# Autodesk Inventor assembly: Bottom_Assembly
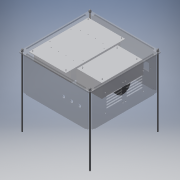
[picture p0: Inventor's stored thumbnail of the model, 180x180]
Saved by Autodesk Inventor 2016 (Build 200138000, 138)
## iProperties
Created: 2018-05-12
Part Number: Bottom_Assembly
Document SubType Name: Assembly
Designer: Phil Erle
Author: Phil Erle
## Documents named in this file (29)
- C:\Users\Phil Erle\Desktop\Adrastea\Bottom_Assembly.iam
- C:\Users\Phil Erle\Desktop\Adrastea\bottom.ipt
- C:\Users\Phil Erle\Desktop\Adrastea\Heatsink.ipt
- C:\Users\Phil Erle\Desktop\Adrastea\Elektronik_Gehäuse.ipt
- C:\Users\Phil Erle\Desktop\Adrastea\GT175DA120U.ipt
- C:\Users\Phil Erle\Desktop\Adrastea\SeitenUntenHinten.ipt
- C:\Users\Phil Erle\Desktop\Adrastea\SeitenUnten.ipt
- C:\Users\Phil Erle\Desktop\Adrastea\SeitenUntenVorne.ipt
- C:\Users\Phil Erle\Desktop\Adrastea\SeitenOben.ipt
- C:\Users\Phil Erle\Desktop\Adrastea\mid.ipt
- C:\Users\Phil Erle\Desktop\Adrastea\Main.ipt
- C:\Users\Phil Erle\Desktop\Adrastea\Primary.ipt
- C:\Users\Phil Erle\Desktop\Adrastea\Normteile\Muttern\din1587-m5x0_8ricu3.ipt
- C:\Users\Phil Erle\Desktop\Adrastea\Seconday_End_Bottom.ipt
- C:\Users\Phil Erle\Desktop\Adrastea\M5 Gewindestange.ipt
- C:\Users\Phil Erle\Desktop\Adrastea\Normteile\Muttern\mutter_din934_m5-6.ipt
- C:\Users\Phil Erle\Desktop\Adrastea\Secondary.ipt
- C:\Users\Phil Erle\Desktop\Adrastea\TopLoad.ipt
- C:\Users\Phil Erle\Desktop\Adrastea\Seconday_End_Top.ipt
- C:\Users\Phil Erle\Desktop\Adrastea\M6 Gewindestange.ipt
- C:\Users\Phil Erle\Desktop\Adrastea\top.ipt
- C:\Users\Phil Erle\Desktop\Adrastea\Coil.ipt
- C:\Users\Phil Erle\Desktop\Adrastea\primary_holder.ipt
- C:\Users\Phil Erle\Desktop\Adrastea\IGBT_Platine.ipt
- C:\Users\Phil Erle\Desktop\Adrastea\Cap_Holder_1.ipt
- C:\Users\Phil Erle\Desktop\Adrastea\Cap.ipt
- C:\Users\Phil Erle\Desktop\Adrastea\Abstandshalter_10mm_M4.ipt
- C:\Users\Phil Erle\Desktop\Adrastea\CU5.ipt
- C:\Users\Phil Erle\Desktop\Adrastea\Snubber.ipt
## Components (50 placed, 28 different names)
1. bottom:1 — Mate:1, Mate:2, Flush:1, Mate:3, Mate:4, Mate:5, Mate:6, Mate:7, Mate:8, Mate:21, Mate:24, Mate:25, Mate:27, Mate:31, Mate:32, Mate:36, Mate:37, Mate:38, Mate:39, Mate:40, Mate:41, Mate:60, Mate:61, Mate:62, Mate:63, Mate:64, Mate:65, Mate:66, Mate:67, Mate:68, Mate:69, Mate:70, Mate:71, Flush:2, Flush:3, Flush:4, Flush:5
2. Heatsink:1 — Mate:3, Mate:4, Mate:5, Mate:9, Mate:10, Mate:11, Mate:12, Mate:13, Mate:14, Mate:15, Mate:16, Mate:17, Mate:18, Mate:19, Mate:20, Mate:106, Mate:107
3. Elektronik_Gehäuse:1 — Mate:6, Mate:7, Mate:8
4. GT175DA120U:1 — Mate:9, Mate:16, Mate:20, Mate:103, Mate:104, Mate:105, Mate:109, Mate:110, Mate:111
5. GT175DA120U:2 — Mate:10, Mate:14, Mate:19
6. GT175DA120U:3 — Mate:11, Mate:15, Mate:18
7. GT175DA120U:4 — Mate:12, Mate:13, Mate:17
8. SeitenUntenHinten:1 — Mate:21, Mate:27, Mate:31, Mate:34
9. SeitenUnten:1 — Mate:36, Mate:37, Mate:38
10. SeitenUnten:2 — Mate:24, Mate:25, Mate:32, Mate:43
11. SeitenUntenVorne:1 — Mate:39, Mate:40, Mate:41, Mate:42, Mate:44
12. SeitenOben:1 — Mate:45, Mate:51, Mate:56, Mate:59
13. SeitenOben:2 — Mate:46, Mate:52, Mate:53, Mate:58
14. SeitenOben:3 — Mate:48, Mate:49, Mate:55, Mate:57
15. SeitenOben:4 — Mate:47, Mate:50, Mate:54
16. mid:1 — Mate:34, Mate:42, Mate:43, Mate:44, Mate:45, Mate:46, Mate:47, Mate:48, Mate:49, Mate:50, Mate:51, Mate:52, Mate:53, Mate:54, Mate:55, Mate:56
17. Main:1 — Mate:57, Mate:58, Mate:59, Mate:72, Mate:73, Mate:75, Mate:76, Mate:77, Mate:85, Mate:86, Mate:87, Mate:88, Mate:92
18. Primary:1 — Mate:89, Mate:90, Mate:91
19. din1587-m5x0_8ricu3:1 — Mate:62, Mate:65
20. din1587-m5x0_8ricu3:2 — Mate:63, Mate:67
21. din1587-m5x0_8ricu3:3 — Mate:60, Mate:66
22. din1587-m5x0_8ricu3:4 — Mate:61, Mate:64
23. Seconday_End_Bottom:1 — Mate:72, Mate:92, Mate:93, Mate:94
24. M5 Gewindestange:1 — Mate:68, Flush:3, Mate:78, Mate:83
25. M5 Gewindestange:2 — Mate:70, Flush:4, Mate:80, Mate:82, Mate:90
26. M5 Gewindestange:3 — Mate:69, Flush:2, Mate:79, Mate:84
27. M5 Gewindestange:4 — Mate:71, Flush:5, Mate:74, Mate:81, Mate:91
28. mutter_din934_m5-6:1 — Mate:73, Mate:74
29. mutter_din934_m5-6:2 — Mate:75, Mate:80
30. mutter_din934_m5-6:3 — Mate:77, Mate:78
31. mutter_din934_m5-6:4 — Mate:76, Mate:79
32. mutter_din934_m5-6:5 — Mate:82, Mate:86
33. mutter_din934_m5-6:6 — Mate:83, Mate:88
34. mutter_din934_m5-6:7 — Mate:84, Mate:85
35. mutter_din934_m5-6:8 — Mate:81, Mate:87, Mate:89
36. Secondary:1 — Mate:93, Mate:94, Mate:95, Mate:96, Mate:102, Flush:7
37. TopLoad:1 — Mate:98, Mate:99, Flush:6
38. Seconday_End_Top:1 — Mate:95, Mate:96, Mate:97, Mate:99
39. M6 Gewindestange:1 — Mate:97, Mate:98, Mate:100, Mate:101
40. top:1 — Mate:100, Flush:6, Mate:101
41. Coil:1 — Mate:102, Flush:7
42. primary_holder:1
43. IGBT_Platine:1 — Mate:103, Mate:104, Mate:105, Mate:112, Mate:113, Mate:114
44. Cap_Holder_1:1 — Mate:106, Mate:107, Mate:108, Flush:8
45. Cap:1 — Mate:108, Flush:8
46. Abstandshalter_10mm_M4:1 — Mate:111, Mate:113, Mate:117
47. Abstandshalter_10mm_M4:2 — Mate:110, Mate:114, Mate:115
48. Abstandshalter_10mm_M4:3 — Mate:109, Mate:112, Mate:116
49. CU5:1 — Mate:115, Mate:116, Mate:117, Mate:118
50. Snubber:1 — Mate:118
## Relationships (118: Mate 110, Flush 8)
- Mate:1: bottom:1
- Mate:2: bottom:1
- Flush:1: bottom:1
- Mate:3: bottom:1 ↔ Heatsink:1
- Mate:4: bottom:1 ↔ Heatsink:1
- Mate:5: bottom:1 ↔ Heatsink:1
- Mate:6: bottom:1 ↔ Elektronik_Gehäuse:1
- Mate:7: bottom:1 ↔ Elektronik_Gehäuse:1
- Mate:8: bottom:1 ↔ Elektronik_Gehäuse:1
- Mate:9: Heatsink:1 ↔ GT175DA120U:1
- Mate:10: Heatsink:1 ↔ GT175DA120U:2
- Mate:11: Heatsink:1 ↔ GT175DA120U:3
- Mate:12: Heatsink:1 ↔ GT175DA120U:4
- Mate:13: Heatsink:1 ↔ GT175DA120U:4
- Mate:14: Heatsink:1 ↔ GT175DA120U:2
- Mate:15: Heatsink:1 ↔ GT175DA120U:3
- Mate:16: Heatsink:1 ↔ GT175DA120U:1
- Mate:17: Heatsink:1 ↔ GT175DA120U:4
- Mate:18: Heatsink:1 ↔ GT175DA120U:3
- Mate:19: Heatsink:1 ↔ GT175DA120U:2
- Mate:20: Heatsink:1 ↔ GT175DA120U:1
- Mate:21: bottom:1 ↔ SeitenUntenHinten:1
- Mate:24: bottom:1 ↔ SeitenUnten:2
- Mate:25: bottom:1 ↔ SeitenUnten:2
- Mate:27: bottom:1 ↔ SeitenUntenHinten:1
- Mate:31: bottom:1 ↔ SeitenUntenHinten:1
- Mate:32: bottom:1 ↔ SeitenUnten:2
- Mate:34: SeitenUntenHinten:1 ↔ mid:1
- Mate:36: bottom:1 ↔ SeitenUnten:1
- Mate:37: bottom:1 ↔ SeitenUnten:1
- Mate:38: bottom:1 ↔ SeitenUnten:1
- Mate:39: bottom:1 ↔ SeitenUntenVorne:1
- Mate:40: bottom:1 ↔ SeitenUntenVorne:1
- Mate:41: bottom:1 ↔ SeitenUntenVorne:1
- Mate:42: SeitenUntenVorne:1 ↔ mid:1
- Mate:43: SeitenUnten:2 ↔ mid:1
- Mate:44: SeitenUntenVorne:1 ↔ mid:1
- Mate:45: SeitenOben:1 ↔ mid:1
- Mate:46: SeitenOben:2 ↔ mid:1
- Mate:47: SeitenOben:4 ↔ mid:1
- Mate:48: SeitenOben:3 ↔ mid:1
- Mate:49: SeitenOben:3 ↔ mid:1
- Mate:50: SeitenOben:4 ↔ mid:1
- Mate:51: SeitenOben:1 ↔ mid:1
- Mate:52: SeitenOben:2 ↔ mid:1
- Mate:53: SeitenOben:2 ↔ mid:1
- Mate:54: SeitenOben:4 ↔ mid:1
- Mate:55: SeitenOben:3 ↔ mid:1
- Mate:56: SeitenOben:1 ↔ mid:1
- Mate:57: SeitenOben:3 ↔ Main:1
- Mate:58: SeitenOben:2 ↔ Main:1
- Mate:59: SeitenOben:1 ↔ Main:1
- Mate:60: bottom:1 ↔ din1587-m5x0_8ricu3:3
- Mate:61: bottom:1 ↔ din1587-m5x0_8ricu3:4
- Mate:62: bottom:1 ↔ din1587-m5x0_8ricu3:1
- Mate:63: bottom:1 ↔ din1587-m5x0_8ricu3:2
- Mate:64: bottom:1 ↔ din1587-m5x0_8ricu3:4
- Mate:65: bottom:1 ↔ din1587-m5x0_8ricu3:1
- Mate:66: bottom:1 ↔ din1587-m5x0_8ricu3:3
- Mate:67: bottom:1 ↔ din1587-m5x0_8ricu3:2
- Mate:68: bottom:1 ↔ M5 Gewindestange:1
- Mate:69: bottom:1 ↔ M5 Gewindestange:3
- Mate:70: bottom:1 ↔ M5 Gewindestange:2
- Mate:71: bottom:1 ↔ M5 Gewindestange:4
- Mate:72: Main:1 ↔ Seconday_End_Bottom:1
- Flush:2 (-3 mm): bottom:1 ↔ M5 Gewindestange:3
- Flush:3 (-3 mm): bottom:1 ↔ M5 Gewindestange:1
- Flush:4 (-3 mm): bottom:1 ↔ M5 Gewindestange:2
- Flush:5 (-3 mm): bottom:1 ↔ M5 Gewindestange:4
- Mate:73: Main:1 ↔ mutter_din934_m5-6:1
- Mate:74: M5 Gewindestange:4 ↔ mutter_din934_m5-6:1
- Mate:75: Main:1 ↔ mutter_din934_m5-6:2
- Mate:76: Main:1 ↔ mutter_din934_m5-6:4
- Mate:77: Main:1 ↔ mutter_din934_m5-6:3
- Mate:78: M5 Gewindestange:1 ↔ mutter_din934_m5-6:3
- Mate:79: M5 Gewindestange:3 ↔ mutter_din934_m5-6:4
- Mate:80: M5 Gewindestange:2 ↔ mutter_din934_m5-6:2
- Mate:81: M5 Gewindestange:4 ↔ mutter_din934_m5-6:8
- Mate:82: M5 Gewindestange:2 ↔ mutter_din934_m5-6:5
- Mate:83: M5 Gewindestange:1 ↔ mutter_din934_m5-6:6
- Mate:84: M5 Gewindestange:3 ↔ mutter_din934_m5-6:7
- Mate:85 (40 mm): Main:1 ↔ mutter_din934_m5-6:7
- Mate:86 (40 mm): Main:1 ↔ mutter_din934_m5-6:5
- Mate:87 (40 mm): Main:1 ↔ mutter_din934_m5-6:8
- Mate:88 (40 mm): Main:1 ↔ mutter_din934_m5-6:6
- Mate:89: Primary:1 ↔ mutter_din934_m5-6:8
- Mate:90: Primary:1 ↔ M5 Gewindestange:2
- Mate:91: Primary:1 ↔ M5 Gewindestange:4
- Mate:92: Main:1 ↔ Seconday_End_Bottom:1
- Mate:93: Seconday_End_Bottom:1 ↔ Secondary:1
- Mate:94: Seconday_End_Bottom:1 ↔ Secondary:1
- Mate:95: Secondary:1 ↔ Seconday_End_Top:1
- Mate:96: Secondary:1 ↔ Seconday_End_Top:1
- Mate:97: Seconday_End_Top:1 ↔ M6 Gewindestange:1
- Mate:98: TopLoad:1 ↔ M6 Gewindestange:1
- Mate:99 (150 mm): TopLoad:1 ↔ Seconday_End_Top:1
- Mate:100: M6 Gewindestange:1 ↔ top:1
- Flush:6 (150 mm): TopLoad:1 ↔ top:1
- Mate:101 (-5 mm): M6 Gewindestange:1 ↔ top:1
- Mate:102: Secondary:1 ↔ Coil:1
- Flush:7 (-50 mm): Secondary:1 ↔ Coil:1
- Mate:103: GT175DA120U:1 ↔ IGBT_Platine:1
- Mate:104: GT175DA120U:1 ↔ IGBT_Platine:1
- Mate:105: GT175DA120U:1 ↔ IGBT_Platine:1
- Mate:106: Heatsink:1 ↔ Cap_Holder_1:1
- Mate:107: Heatsink:1 ↔ Cap_Holder_1:1
- Mate:108: Cap_Holder_1:1 ↔ Cap:1
- Flush:8: Cap_Holder_1:1 ↔ Cap:1
- Mate:109: GT175DA120U:1 ↔ Abstandshalter_10mm_M4:3
- Mate:110: GT175DA120U:1 ↔ Abstandshalter_10mm_M4:2
- Mate:111: GT175DA120U:1 ↔ Abstandshalter_10mm_M4:1
- Mate:112: IGBT_Platine:1 ↔ Abstandshalter_10mm_M4:3
- Mate:113: IGBT_Platine:1 ↔ Abstandshalter_10mm_M4:1
- Mate:114: IGBT_Platine:1 ↔ Abstandshalter_10mm_M4:2
- Mate:115: Abstandshalter_10mm_M4:2 ↔ CU5:1
- Mate:116: Abstandshalter_10mm_M4:3 ↔ CU5:1
- Mate:117: Abstandshalter_10mm_M4:1 ↔ CU5:1
- Mate:118: CU5:1 ↔ Snubber:1
